# Autodesk Inventor assembly: cross_frame_axle
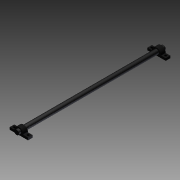
[picture p0: Inventor's stored thumbnail of the model, 180x180]
Saved by Autodesk Inventor 2011 (Build 150239000, 239)
## iProperties
Created: 2013-01-19
Part Number: cross_frame_axle
Document SubType Name: Assembly
Designer: Christopher
Author: Christopher
## Documents named in this file (3)
- F:\Users\Christopher\Documents\GitHub\2013CAD\2013 robot\forklift\Pneumatics and frame grabbers\cross_frame_axle.iam
- F:\Users\Christopher\Documents\GitHub\2013CAD\2013 robot\forklift\Misc parts\.5inch_side_bearing.ipt
- F:\Users\Christopher\Documents\GitHub\2013CAD\2013 robot\forklift\Pneumatics and frame grabbers\cross_mid_frame_axle.ipt
## Components (3 placed, 2 different names)
1. .5inch_side_bearing:1 — Insert:1, Flush:1
2. cross_mid_frame_axle:1 — Insert:1, Insert:2
3. .5inch_side_bearing:2 — Insert:2, Flush:1
## Relationships (3: Insert 2, Flush 1)
- Insert:1 (6.35 mm): .5inch_side_bearing:1 ↔ cross_mid_frame_axle:1
- Insert:2 (6.35 mm): cross_mid_frame_axle:1 ↔ .5inch_side_bearing:2
- Flush:1: .5inch_side_bearing:1 ↔ .5inch_side_bearing:2
